# Autodesk Inventor assembly: CC1x1
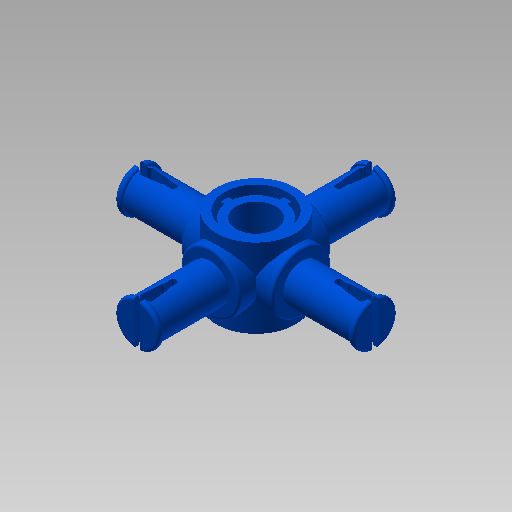
[picture p0: Inventor's stored thumbnail of the model, 512x512]
Saved by Autodesk Inventor 2019.3 (Build 233278000, 278)
## iProperties
Created: 2019-02-06
Part Number: CC1x1
Document SubType Name: Assembly
Designer: Varga Daniel
Author: Varga Daniel
## Documents named in this file (5)
- C:\!_Dani\!_cloud\OneDrive\!_munka\Revolution\RevvyDemoKit\Structural parts\Connector Boxes\Connector cubes\CC1x1.iam
- C:\!_Dani\!_cloud\OneDrive\!_munka\Revolution\RevvyDemoKit\Structural parts\Connetor Pins\Connector_pin_stick.ipt
- C:\!_Dani\!_cloud\OneDrive\!_munka\Revolution\RevvyDemoKit\Structural parts\Connector Boxes\Connector_box_collar.ipt
- C:\!_Dani\!_cloud\OneDrive\!_munka\Revolution\RevvyDemoKit\Structural parts\Connector Boxes\Connector_box_single_part.ipt
- C:\!_Dani\!_cloud\OneDrive\!_munka\Revolution\RevvyDemoKit\Structural parts\Connector Boxes\Connector_box_collar\Connector_box_collar-both.ipt
## Components (9 placed, 3 different names)
1. Connector_pin_stick:1 — Mate:1, Mate:2, Mate:16, Angle:2
2. Connector_box_single_part:1 — Mate:9, Mate:10, Mate:11, Mate:12, Mate:13, Mate:14, Mate:15, Mate:16, Mate:17
3. Connector_box_collar-both:1 — Mate:1, Mate:2, Mate:9
4. Connector_pin_stick:2 — Mate:14, Angle:4
5. Connector_box_collar-both:2 — Mate:12
6. Connector_pin_stick:3 — Mate:15, Angle:1, Angle:2
7. Connector_box_collar-both:3 — Mate:11, Angle:3
8. Connector_pin_stick:4 — Mate:13, Angle:3, Angle:4
9. Connector_box_collar-both:4 — Mate:10, Angle:1
## Relationships (21: Mate 17, Angle 4)
- Mate:1: Connector_pin_stick:1 ↔ Connector_box_collar-both:1
- Mate:2: Connector_pin_stick:1 ↔ Connector_box_collar-both:1
- [Mate]: Connector_pin_stick:2 ↔ Connector_box_collar-both:2
- [Mate]: Connector_pin_stick:2 ↔ Connector_box_collar-both:2
- [Mate]: Connector_pin_stick:3 ↔ Connector_box_collar-both:3
- [Mate]: Connector_pin_stick:3 ↔ Connector_box_collar-both:3
- [Mate]: Connector_pin_stick:4 ↔ Connector_box_collar-both:4
- [Mate]: Connector_pin_stick:4 ↔ Connector_box_collar-both:4
- Mate:9: Connector_box_single_part:1 ↔ Connector_box_collar-both:1
- Mate:10: Connector_box_single_part:1 ↔ Connector_box_collar-both:4
- Mate:11: Connector_box_single_part:1 ↔ Connector_box_collar-both:3
- Mate:12: Connector_box_single_part:1 ↔ Connector_box_collar-both:2
- Mate:13: Connector_box_single_part:1 ↔ Connector_pin_stick:4
- Mate:14: Connector_box_single_part:1 ↔ Connector_pin_stick:2
- Mate:15: Connector_box_single_part:1 ↔ Connector_pin_stick:3
- Mate:16: Connector_pin_stick:1 ↔ Connector_box_single_part:1
- Angle:1 (0 deg): Connector_pin_stick:3 ↔ Connector_box_collar-both:4
- Angle:2 (0 deg): Connector_pin_stick:1 ↔ Connector_pin_stick:3
- Mate:17: Connector_box_single_part:1
- Angle:3 (0 deg): Connector_box_collar-both:3 ↔ Connector_pin_stick:4
- Angle:4 (0 deg): Connector_pin_stick:2 ↔ Connector_pin_stick:4
## Named parameters: d2_d0 = 0 mm, d3_d1 = 0 mm, d4_d0 = 0 mm, d5_d1 = 0 mm, d6_d0 = 0 mm, d7_d1 = 0 mm
